# Autodesk Inventor assembly: Assembly2
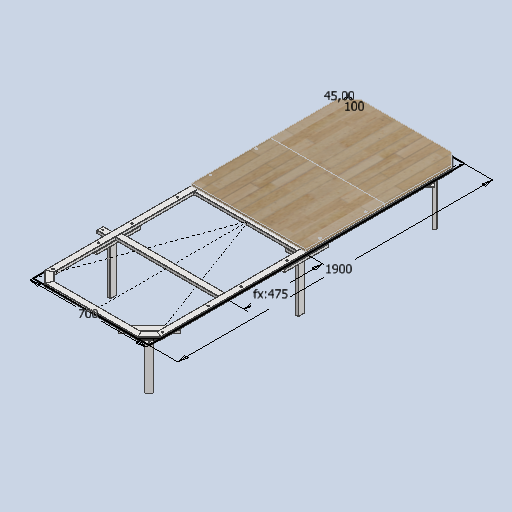
[picture p0: Inventor's stored thumbnail of the model, 512x512]
Saved by Autodesk Inventor 2026.2 (Build 302298000, 298)
## iProperties
Created: 2026-05-20
Part Number: Assembly2
Document SubType Name: Assembly
Designer: admin
Mass: 11655.6 g
Surface Area: 14897.7 cm^2
Volume: 1484.79 cm^3
Density: 7.85 g/cm^3
Author: admin
## Documents named in this file (9)
- C:\Users\admin\Documents\Inventor\Debbed\Assembly2.iam
- C:\Users\admin\Documents\Inventor\Debbed\DBD Dim sketch.ipt
- C:\Users\admin\Documents\Inventor\Debbed\фанера1.ipt
- C:\Users\admin\Documents\Inventor\Debbed\фанера 2.ipt
- C:\Users\admin\Documents\Inventor\Debbed\Long tube 1.ipt
- C:\Users\admin\Documents\Inventor\Debbed\Long tube 1_CPY.ipt
- C:\Users\admin\Documents\Inventor\Debbed\Short tube 2.ipt
- C:\Users\admin\Documents\Inventor\Debbed\Short tube 3.ipt
- C:\Users\admin\Documents\Inventor\Debbed\Assembly Leg.iam
## Components (18 placed, 8 different names)
1. DBD Dim sketch:1 — Mate:3, Mate:6, Mate:13, Mate:16
2. фанера1:1 — Mate:2, Mate:3, Mate:7
3. фанера 2:1 — Flush:4, Mate:17
4. Long tube 1:1 — Flush:2, Mate:6, Flush:3, Rigid:1, Mate:7, Rigid:10, Flush:12
5. Short tube 1:1 — Rigid:2, Rigid:9, Mate:20
6. Short tube 2:1 — Rigid:1, Rigid:2
7. Short tube 3:1 — Mate:8, Mate:9, Mate:10
8. Short tube 2:2 — Rigid:10, Rigid:11
9. Short tube 2:3 — Rigid:12, Rigid:13, Flush:11, Mate:23
10. Short tube 2:4 — Rigid:9, Mate:19, Flush:9, Mate:22
11. Short tube 1:2 — Rigid:11, Rigid:12
12. Long tube 1:2 — Mate:17, Mate:21, Flush:8, Rigid:13
13. Short tube 3:2 — Mate:11, Mate:12, Mate:13, Flush:13
14. Short tube 3:3 — Mate:14, Mate:15, Mate:16
15. Assembly Leg:1 [sub-assembly] — Flush:11, Mate:23
16. Assembly Leg:2 [sub-assembly] — Mate:21, Flush:8
17. Assembly Leg:3 [sub-assembly] — Mate:19, Flush:9, Mate:22
18. Assembly Leg:4 [sub-assembly] — Mate:20, Flush:12, Flush:13
## Relationships (35: Mate 20, Flush 8, WeldJoint 7)
- Mate:2: фанера1:1
- Mate:3: DBD Dim sketch:1 ↔ фанера1:1
- Flush:2: Long tube 1:1
- Mate:6: DBD Dim sketch:1 ↔ Long tube 1:1
- Flush:3: Long tube 1:1
- Rigid:1 [WeldJoint]: Long tube 1:1 ↔ Short tube 2:1
- Rigid:2 [WeldJoint]: Short tube 1:1 ↔ Short tube 2:1
- Mate:7: фанера1:1 ↔ Long tube 1:1
- Rigid:9 [WeldJoint]: Short tube 1:1 ↔ Short tube 2:4
- Mate:8: Short tube 3:1
- Mate:9: Short tube 3:1
- Mate:10: Short tube 3:1
- Mate:11: Short tube 3:2
- Mate:12: Short tube 3:2
- Mate:13: DBD Dim sketch:1 ↔ Short tube 3:2
- Mate:14: Short tube 3:3
- Mate:15: Short tube 3:3
- Mate:16: DBD Dim sketch:1 ↔ Short tube 3:3
- Flush:4: фанера 2:1
- Mate:17: фанера 2:1 ↔ Long tube 1:2
- [Mate]: Long tube 1:2 ↔ Assembly Leg:1
- Mate:19: Short tube 2:4 ↔ Assembly Leg:3
- Mate:20: Short tube 1:1 ↔ Assembly Leg:4
- Mate:21: Long tube 1:2 ↔ Assembly Leg:2
- Flush:8: Long tube 1:2 ↔ Assembly Leg:2
- Flush:9 (5 mm): Short tube 2:4 ↔ Assembly Leg:3
- Mate:22: Short tube 2:4 ↔ Assembly Leg:3
- Rigid:10 [WeldJoint]: Long tube 1:1 ↔ Short tube 2:2
- Rigid:11 [WeldJoint]: Short tube 2:2 ↔ Short tube 1:2
- Rigid:12 [WeldJoint]: Short tube 2:3 ↔ Short tube 1:2
- Rigid:13 [WeldJoint]: Short tube 2:3 ↔ Long tube 1:2
- Flush:11 (5 mm): Short tube 2:3 ↔ Assembly Leg:1
- Mate:23: Short tube 2:3 ↔ Assembly Leg:1
- Flush:12: Long tube 1:1 ↔ Assembly Leg:4
- Flush:13: Short tube 3:2 ↔ Assembly Leg:4
